# Autodesk Inventor assembly: Leadscrew Bearing Assembly
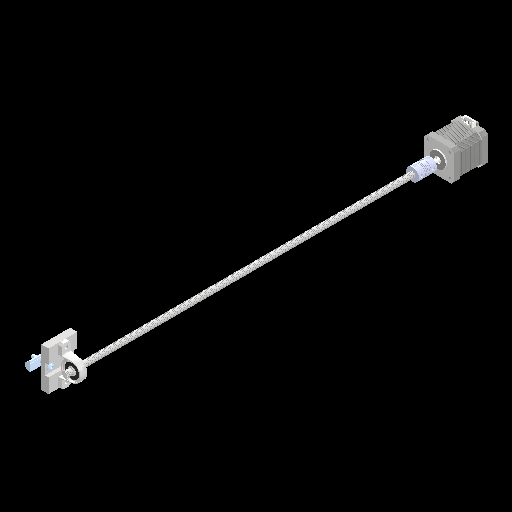
[picture p0: Inventor's stored thumbnail of the model, 512x512]
Saved by Autodesk Inventor 2026.1 (Build 301233000, 233)
## iProperties
Created: 2024-12-30
Part Number: Leadscrew Bearing Assembly
Document SubType Name: Assembly
Designer: drago
Author: drago
## Documents named in this file (7)
- C:\Users\drago\Desktop\_QIST4500_Multidisciplinary_Team_Project\Proteox MX magnet positioner CAD\z_translator\z_translator.iam
- C:\Users\drago\Desktop\_QIST4500_Multidisciplinary_Team_Project\Proteox MX magnet positioner CAD\z_translator\5X8_COUPLER.ipt
- C:\Users\drago\Desktop\_QIST4500_Multidisciplinary_Team_Project\Proteox MX magnet positioner CAD\z_translator\item_61953_t-slot-slider-8-80x40-fa__high.ipt
- C:\Users\drago\Desktop\_QIST4500_Multidisciplinary_Team_Project\Proteox MX magnet positioner CAD\z_translator\KP08.iam
- C:\Users\drago\Desktop\_QIST4500_Multidisciplinary_Team_Project\Proteox MX magnet positioner CAD\z_translator\Leadscrew Bearing Bracket.ipt
- C:\Users\drago\Desktop\_QIST4500_Multidisciplinary_Team_Project\Proteox MX magnet positioner CAD\z_translator\Lead Screw 8mm-2.0 x 500mm.ipt
- C:\Users\drago\Desktop\_QIST4500_Multidisciplinary_Team_Project\Proteox MX magnet positioner CAD\z_translator\Stepper Motor Nema 17.ipt
## Components (7 placed, 6 different names)
1. 5X8_COUPLER:1 — Mate:11, Mate:14, Mate:16, Mate:20
2. item_61953_t-slot-slider-8-80x40-fa__high:1 — Mate:5, Mate:7, Angle:3
3. item_61953_t-slot-slider-8-80x40-fa__high:2 — Mate:4, Mate:6, Angle:2
4. KP08:1 [sub-assembly] — Mate:8, Mate:9, Mate:10, Mate:12, Mate:13
5. Leadscrew Bearing Bracket:1 — Mate:4, Mate:5, Mate:6, Mate:7, Mate:8, Mate:9, Mate:10, Angle:1
6. Lead Screw 8mm-2.0 x 500mm:1 — Mate:11, Mate:12, Mate:13, Mate:15, Mate:19
7. Stepper Motor Nema 17:1 — Mate:14, Mate:15, Mate:16, Mate:17, Mate:18, Angle:1
## Relationships (20: Mate 17, Angle 3)
- Mate:4: item_61953_t-slot-slider-8-80x40-fa__high:2 ↔ Leadscrew Bearing Bracket:1
- Mate:5: item_61953_t-slot-slider-8-80x40-fa__high:1 ↔ Leadscrew Bearing Bracket:1
- Mate:6: item_61953_t-slot-slider-8-80x40-fa__high:2 ↔ Leadscrew Bearing Bracket:1
- Mate:7: item_61953_t-slot-slider-8-80x40-fa__high:1 ↔ Leadscrew Bearing Bracket:1
- Mate:8: KP08:1 ↔ Leadscrew Bearing Bracket:1
- Mate:9: KP08:1 ↔ Leadscrew Bearing Bracket:1
- Mate:10: KP08:1 ↔ Leadscrew Bearing Bracket:1
- Mate:11: 5X8_COUPLER:1 ↔ Lead Screw 8mm-2.0 x 500mm:1
- Mate:12: KP08:1 ↔ Lead Screw 8mm-2.0 x 500mm:1
- Mate:13 (-10 mm): KP08:1 ↔ Lead Screw 8mm-2.0 x 500mm:1
- Mate:14: 5X8_COUPLER:1 ↔ Stepper Motor Nema 17:1
- Mate:15: Lead Screw 8mm-2.0 x 500mm:1 ↔ Stepper Motor Nema 17:1
- Mate:16 (10 mm): 5X8_COUPLER:1 ↔ Stepper Motor Nema 17:1
- Mate:17: Stepper Motor Nema 17:1
- Mate:18: Stepper Motor Nema 17:1
- Angle:1 (90 deg): Leadscrew Bearing Bracket:1 ↔ Stepper Motor Nema 17:1
- Mate:19: Lead Screw 8mm-2.0 x 500mm:1
- Angle:2 (180 deg): item_61953_t-slot-slider-8-80x40-fa__high:2
- Angle:3 (0 deg): item_61953_t-slot-slider-8-80x40-fa__high:1
- Mate:20: 5X8_COUPLER:1
